# Autodesk Inventor assembly: leg_press_v4
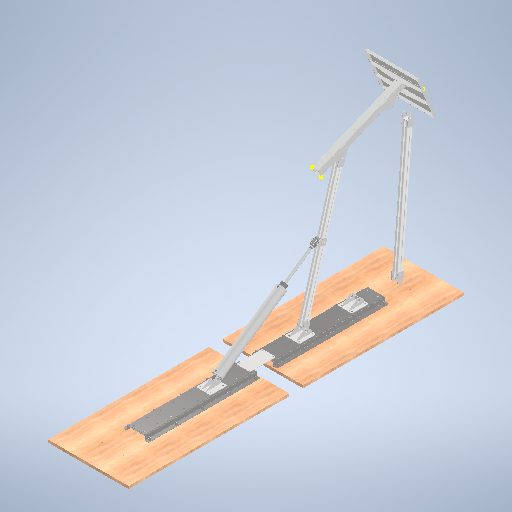
[picture p0: Inventor's stored thumbnail of the model, 512x512]
Saved by Autodesk Inventor 2025.2 (Build 292293000, 293)
## iProperties
Created: 2025-05-02
Part Number: leg_press_v4
Document SubType Name: Assembly
Designer: Caspe
Author: Caspe
## Documents named in this file (11)
- C:\Users\Caspe\Documents\Semester 8\Project\Anomaly_Detection\Mechanical_Project\Inventor_project\leg_press_v4.iam
- C:\Users\Caspe\Documents\Semester 8\Project\Anomaly_Detection\Mechanical_Project\Inventor_project\IMS-00-000_p&g.iam
- C:\Users\Caspe\Documents\Semester 8\Project\Anomaly_Detection\Mechanical_Project\Inventor_project\Extender.ipt
- C:\Users\Caspe\Documents\Semester 8\Project\Anomaly_Detection\Mechanical_Project\Inventor_project\bottom_hinge.iam
- C:\Users\Caspe\Documents\Semester 8\Project\Anomaly_Detection\Mechanical_Project\Inventor_project\A_beam.iam
- C:\Users\Caspe\Documents\Semester 8\Project\Anomaly_Detection\Mechanical_Project\Inventor_project\B_beam.iam
- C:\Users\Caspe\Documents\Semester 8\Project\Anomaly_Detection\Mechanical_Project\Inventor_project\Piston_Bottom_Hinge.iam
- C:\Users\Caspe\Documents\Semester 8\Project\Anomaly_Detection\Mechanical_Project\Inventor_project\193995 DSNU-63-500-P-A---(500PA---00--0-------0).iam
- C:\Users\Caspe\Documents\Semester 8\Project\Anomaly_Detection\Mechanical_Project\Inventor_project\A_B_hinge.ipt
- C:\Users\Caspe\Documents\Semester 8\Project\Anomaly_Detection\Mechanical_Project\Inventor_project\foot pedal.iam
- C:\Users\Caspe\Documents\Semester 8\Project\Anomaly_Detection\Mechanical_Project\Inventor_project\Leg_press_parameters.xlsx
## Components (15 placed, 9 different names)
1. IMS-00-000_p&g:1 [sub-assembly] — Insert:1, Insert:2, Insert:7, Insert:8, Insert:19, Insert:20
2. IMS-00-000_p&g:2 [sub-assembly] — Insert:3, Insert:4, Insert:9, Insert:10
3. Extender:1 — Insert:1, Insert:2, Insert:3, Insert:4
4. bottom_hinge:1 [sub-assembly] — Insert:19, Insert:20
5. A_beam:1 [sub-assembly] — Mate:10
6. bottom_hinge:2 [sub-assembly] — Insert:7, Insert:8, Mate:11, Mate:12
7. A_beam:2 [sub-assembly] — Mate:7, Mate:8, Mate:9, Mate:11, Mate:12
8. B_beam:1 [sub-assembly] — Insert:11, Insert:12, Insert:13, Insert:14, Insert:15, Insert:16, Insert:17, Insert:18, Insert:21, Insert:22
9. Piston_Bottom_Hinge:1 [sub-assembly] — Mate:5, Mate:6, Insert:9, Insert:10
10. 193995 DSNU-63-500-P-A---(500PA---00--0-------0):1 [sub-assembly] — Mate:5, Mate:6, Mate:7
11. A_B_hinge:1 — Mate:8, Insert:11, Insert:12, Mate:9
12. A_B_hinge:2 — Insert:13, Insert:14
13. A_B_hinge:3 — Insert:15, Insert:16, Mate:10
14. A_B_hinge:4 — Insert:17, Insert:18
15. foot pedal:1 [sub-assembly] — Insert:21, Insert:22
## Relationships (28: Insert 20, Mate 8)
- Insert:1: IMS-00-000_p&g:1 ↔ Extender:1
- Insert:2: IMS-00-000_p&g:1 ↔ Extender:1
- Insert:3: IMS-00-000_p&g:2 ↔ Extender:1
- Insert:4: IMS-00-000_p&g:2 ↔ Extender:1
- Insert:7: IMS-00-000_p&g:1 ↔ bottom_hinge:2
- Insert:8: IMS-00-000_p&g:1 ↔ bottom_hinge:2
- Mate:5: Piston_Bottom_Hinge:1 ↔ 193995 DSNU-63-500-P-A---(500PA---00--0-------0):1
- Mate:6 (3 mm): Piston_Bottom_Hinge:1 ↔ 193995 DSNU-63-500-P-A---(500PA---00--0-------0):1
- Insert:9: IMS-00-000_p&g:2 ↔ Piston_Bottom_Hinge:1
- Insert:10: IMS-00-000_p&g:2 ↔ Piston_Bottom_Hinge:1
- Mate:7: A_beam:2 ↔ 193995 DSNU-63-500-P-A---(500PA---00--0-------0):1
- Mate:8: A_beam:2 ↔ A_B_hinge:1
- Insert:11: B_beam:1 ↔ A_B_hinge:1
- Insert:12: B_beam:1 ↔ A_B_hinge:1
- Insert:13: B_beam:1 ↔ A_B_hinge:2
- Insert:14: B_beam:1 ↔ A_B_hinge:2
- Mate:9 (2 mm): A_beam:2 ↔ A_B_hinge:1
- Insert:15: B_beam:1 ↔ A_B_hinge:3
- Insert:16: B_beam:1 ↔ A_B_hinge:3
- Insert:17: B_beam:1 ↔ A_B_hinge:4
- Insert:18: B_beam:1 ↔ A_B_hinge:4
- Mate:10: A_beam:1 ↔ A_B_hinge:3
- Insert:19: IMS-00-000_p&g:1 ↔ bottom_hinge:1
- Insert:20: IMS-00-000_p&g:1 ↔ bottom_hinge:1
- Insert:21: B_beam:1 ↔ foot pedal:1
- Insert:22: B_beam:1 ↔ foot pedal:1
- Mate:11: bottom_hinge:2 ↔ A_beam:2
- Mate:12 (3 mm): bottom_hinge:2 ↔ A_beam:2
## Named parameters: A_length = 1000 mm, A_width = 46 mm, A_bend = 20 mm, A_connection_width = 40 mm, A_displacement = 500 mm, A_hole_height = 10 mm, A_hole_length = 40 mm, A_joint_diameter = 16 mm, A_height = 50 mm, A_B_spacing = 2 mm, A_joint_tolerance = 3 mm, l___________ = 0 mm, B_length = 700 mm, B_height = 50 mm, B_width = 50 mm, B_bend = 20 mm, B_connection_width = 40 mm, B_hole_height = 10 mm, B_hinge_holes_spacing = 50 mm, B_hole_length = 40 mm, l__________ = 0 mm, C_length = 400 mm, C_width = 20 mm, C_height = 330 mm, l_________ = 0 mm, rivet_diameter = 3.35 mm, rivet_displacement = 250 mm, plate_thickness = 3 mm, l________ = 0 mm, L_Piston_Top = 25 mm, L_Piston_Bottom = 21 mm, thin_plate = 1.5 mm
